# Autodesk Inventor assembly: ActualHolderCut
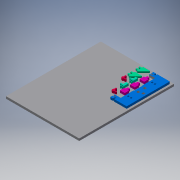
[picture p0: Inventor's stored thumbnail of the model, 180x180]
Saved by Autodesk Inventor 2019 (Build 230136000, 136)
## iProperties
Created: 2018-12-10
Part Number: ActualHolderCut
Document SubType Name: Assembly
Designer: Administrator
Author: Administrator
## Documents named in this file (7)
- H:\Space\Monster Holder\ActualHolderCut.iam
- H:\Space\Monster Holder\CuttingBoardPrint.ipt
- H:\Space\Monster Holder\MonsterHolderSupport1.ipt
- H:\Space\Monster Holder\MonsterHolderSupport3.ipt
- H:\Space\Monster Holder\MonsterSupportHolder4.ipt
- H:\Space\Monster Holder\MonsterHolderBase.ipt
- H:\Space\Monster Holder\switchholder.ipt
## Components (11 placed, 6 different names)
1. CuttingBoardPrint:1 — Mate:1, Mate:2, Mate:3, Mate:4, Mate:5, Mate:6, Mate:7, Mate:8, Mate:9, Mate:10
2. MonsterHolderSupport1:1 — Mate:3
3. MonsterHolderSupport1:2 — Mate:2
4. MonsterHolderSupport3:1 — Mate:7
5. MonsterHolderSupport3:2 — Mate:6
6. MonsterSupportHolder4:1 — Mate:5
7. MonsterSupportHolder4:2 — Mate:4
8. MonsterHolderBase:1 — Mate:1
9. switchholder:1 — Mate:8
10. switchholder:2 — Mate:9
11. switchholder:3 — Mate:10
## Relationships (10: Mate 10)
- Mate:1: CuttingBoardPrint:1 ↔ MonsterHolderBase:1
- Mate:2: CuttingBoardPrint:1 ↔ MonsterHolderSupport1:2
- Mate:3: CuttingBoardPrint:1 ↔ MonsterHolderSupport1:1
- Mate:4: CuttingBoardPrint:1 ↔ MonsterSupportHolder4:2
- Mate:5: CuttingBoardPrint:1 ↔ MonsterSupportHolder4:1
- Mate:6: CuttingBoardPrint:1 ↔ MonsterHolderSupport3:2
- Mate:7: CuttingBoardPrint:1 ↔ MonsterHolderSupport3:1
- Mate:8: CuttingBoardPrint:1 ↔ switchholder:1
- Mate:9: CuttingBoardPrint:1 ↔ switchholder:2
- Mate:10: CuttingBoardPrint:1 ↔ switchholder:3
